# Autodesk Inventor assembly: Pok Mk3
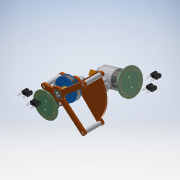
[picture p0: Inventor's stored thumbnail of the model, 180x180]
Saved by Autodesk Inventor 2018.2 (Build 222227000, 227)
## iProperties
Created: 2018-02-12
Part Number: Pok Mk3
Document SubType Name: Assembly
Designer: Moochster
Author: Moochster
## Documents named in this file (19)
- C:\Users\Moochster\OneDrive\Documents\2018 UBC\ELEC 391\Controller\CAD\Pok Mk3.iam
- C:\Users\Moochster\OneDrive\Documents\2018 UBC\ELEC 391\Controller\CAD\Brass Bushing.ipt
- C:\Users\Moochster\OneDrive\Documents\2018 UBC\ELEC 391\Controller\CAD\Rod 3-8in.ipt
- C:\Users\Moochster\OneDrive\Documents\2018 UBC\ELEC 391\Controller\CAD\R1038_ZZ_W Bearing.ipt
- C:\Users\Moochster\OneDrive\Documents\2018 UBC\ELEC 391\Controller\CAD\Yaw Platform Top.ipt
- C:\Users\Moochster\OneDrive\Documents\2018 UBC\ELEC 391\Controller\CAD\Pok Mk3\Design Accelerator\Synchronous Belts Transmission2.iam
- C:\Users\Moochster\OneDrive\Documents\2018 UBC\ELEC 391\Controller\CAD\Pok Header Mount.ipt
- C:\Users\Moochster\OneDrive\Documents\2018 UBC\ELEC 391\Controller\CAD\JD5B-2655W-R.ipt
- C:\Users\Moochster\OneDrive\Documents\2018 UBC\ELEC 391\Controller\CAD\Pok Default Pitch Motor Mount.ipt
- C:\Users\Moochster\OneDrive\Documents\2018 UBC\ELEC 391\Controller\CAD\Laser Mount.ipt
- C:\Users\Moochster\Documents\Inventor\Content Center Files\R2018\en-US\AS 1110\AS 1110 - M3 x 20.ipt
- C:\Users\Moochster\Documents\Inventor\Content Center Files\R2018\en-US\AS 1112 (2)\AS 1112 - M3  Type 5.ipt
- C:\Users\Moochster\Documents\Inventor\Content Center Files\R2018\en-US\CNS 5050\CNS 5050 - A - 3.2 8.ipt
- C:\Users\Moochster\Documents\Inventor\Content Center Files\R2018\en-US\ANSI B18.3.1M(1)\ANSI B18.3.1M - M1.6x0.35 x 3(2).ipt
- C:\Users\Moochster\OneDrive\Documents\2018 UBC\ELEC 391\Controller\CAD\Pok Mk3 Base.ipt
- C:\Users\Moochster\OneDrive\Documents\2018 UBC\ELEC 391\Controller\CAD\Pok Mk3 Support.ipt
- C:\Users\Moochster\OneDrive\Documents\2018 UBC\ELEC 391\Controller\CAD\Encoder Wheel (G16).ipt
- C:\Users\Moochster\OneDrive\Documents\2018 UBC\ELEC 391\Controller\CAD\Shaft Encoder Adapter.ipt
- C:\Users\Moochster\OneDrive\Documents\2018 UBC\ELEC 391\Controller\CAD\GP1A52HRJ00F (Large slot detector).ipt
## Components (34 placed, 18 different names)
1. Brass Bushing:1 — Mate:4, Flush:3, Mate:9
2. Brass Bushing:2 — Mate:3, Mate:8, Mate:31
3. Rod 3-8in:1 — Mate:1, Mate:2, Mate:3, Mate:4, Flush:1, Mate:6, Mate:10, Mate:23, Mate:24, Flush:6
4. R1038_ZZ_W Bearing:1 — Mate:1, Flush:1, Mate:8
5. R1038_ZZ_W Bearing:2 — Mate:2, Mate:5, Flush:2
6. Yaw Platform Top:1 — Mate:5, Flush:2, Flush:3, Mate:11, Angle:1
7. Synchronous Belts Transmission:1 [sub-assembly] — Mate:6, Mate:9, Mate:31, Mate:33
8. Pok Header Mount:1 — Mate:10, Mate:11, Mate:12, Flush:4, Mate:19, Mate:20, Mate:21
9. R1038_ZZ_W Bearing:3 — Mate:12, Flush:4
10. JD5B-2655W-R:1 — Mate:17, Mate:18, Mate:22, Flush:5, Angle:2, Tangent:1, Tangent:2, Mate:34, Mate:38
11. Laser Mount:1 — Mate:17, Mate:18
12. Pok Default Pitch Motor Mount:1 — Mate:19, Mate:20, Mate:21, Mate:22, Flush:5, Mate:25, Insert:1, Insert:3, Insert:5, Insert:7, Angle:2, Mate:26, Mate:27
13. AS 1110 - Metric M3 x 20:1 — Mate:25, Insert:2
14. AS 1110 - Metric M3 x 20:2 — Insert:6
15. CNS 5050 A - 3.2:4 — Insert:7, Insert:8
16. CNS 5050 A - 3.2:2 — Insert:5, Insert:6
17. CNS 5050 A - 3.2:3 — Insert:3, Insert:4
18. CNS 5050 A - 3.2:1 — Insert:1, Insert:2
19. AS 1112 (2) - Metric M3  Type 5:1 — Insert:8
20. AS 1112 (2) - Metric M3  Type 5:2 — Insert:4
21. Broached Socket Head Cap Screw - Metric M1.6x0.35 x 3:1 — Mate:26, Tangent:1
22. Broached Socket Head Cap Screw - Metric M1.6x0.35 x 3:2 — Mate:27, Tangent:2
23. Pok Mk3 Base:1 — Flush:6, Mate:28, Flush:7, Mate:29, Flush:8, Mate:30, Flush:9
24. Pok Mk3 Support:1 — Mate:28, Flush:7
25. Pok Mk3 Support:2 — Mate:30, Flush:9
26. Pok Mk3 Support:3 — Mate:29, Flush:8
27. JD5B-2655W-R:2 — Mate:32, Mate:33
28. Encoder Wheel (G16):1 — Mate:32
29. Encoder Wheel (G16):2 — Mate:35, Mate:36, Mate:37
30. Shaft Encoder Adapter:1 — Mate:34, Mate:35, Mate:36, Mate:37, Mate:38
31. GP1A52HRJ00F (Large slot detector):1
32. GP1A52HRJ00F (Large slot detector):2
33. GP1A52HRJ00F (Large slot detector):3
34. GP1A52HRJ00F (Large slot detector):4
## Relationships (54: Mate 33, Flush 9, Insert 8, Angle 2, Tangent 2)
- Mate:1: Rod 3-8in:1 ↔ R1038_ZZ_W Bearing:1
- Mate:2: Rod 3-8in:1 ↔ R1038_ZZ_W Bearing:2
- Mate:3: Brass Bushing:2 ↔ Rod 3-8in:1
- Mate:4: Brass Bushing:1 ↔ Rod 3-8in:1
- Flush:1: Rod 3-8in:1 ↔ R1038_ZZ_W Bearing:1
- Mate:5: R1038_ZZ_W Bearing:2 ↔ Yaw Platform Top:1
- Flush:2: R1038_ZZ_W Bearing:2 ↔ Yaw Platform Top:1
- Mate:6: Rod 3-8in:1 ↔ Synchronous Belts Transmission:1
- Mate:8 (0.1 mm): Brass Bushing:2 ↔ R1038_ZZ_W Bearing:1
- Flush:3 (0.1 mm): Brass Bushing:1 ↔ Yaw Platform Top:1
- Mate:9 (0.1 mm): Brass Bushing:1 ↔ Synchronous Belts Transmission:1
- Mate:10: Rod 3-8in:1 ↔ Pok Header Mount:1
- Mate:11 (0.2 mm): Yaw Platform Top:1 ↔ Pok Header Mount:1
- Mate:12: Pok Header Mount:1 ↔ R1038_ZZ_W Bearing:3
- Flush:4 (1 mm): Pok Header Mount:1 ↔ R1038_ZZ_W Bearing:3
- Mate:17: JD5B-2655W-R:1 ↔ Laser Mount:1
- Mate:18 (1 mm): JD5B-2655W-R:1 ↔ Laser Mount:1
- Mate:19: Pok Header Mount:1 ↔ Pok Default Pitch Motor Mount:1
- Mate:20: Pok Header Mount:1 ↔ Pok Default Pitch Motor Mount:1
- Mate:21 (0.1 mm): Pok Header Mount:1 ↔ Pok Default Pitch Motor Mount:1
- Mate:22: JD5B-2655W-R:1 ↔ Pok Default Pitch Motor Mount:1
- Mate:23: Rod 3-8in:1
- Mate:24: Rod 3-8in:1
- Angle:1 (0 deg): Yaw Platform Top:1
- Flush:5 (-10 mm): JD5B-2655W-R:1 ↔ Pok Default Pitch Motor Mount:1
- Mate:25: Pok Default Pitch Motor Mount:1 ↔ AS 1110 - Metric M3 x 20:1
- Insert:1: Pok Default Pitch Motor Mount:1 ↔ CNS 5050 A - 3.2:1
- Insert:2: AS 1110 - Metric M3 x 20:1 ↔ CNS 5050 A - 3.2:1
- Insert:3: Pok Default Pitch Motor Mount:1 ↔ CNS 5050 A - 3.2:3
- Insert:4: CNS 5050 A - 3.2:3 ↔ AS 1112 (2) - Metric M3  Type 5:2
- Insert:5: Pok Default Pitch Motor Mount:1 ↔ CNS 5050 A - 3.2:2
- Insert:6: AS 1110 - Metric M3 x 20:2 ↔ CNS 5050 A - 3.2:2
- Insert:7: Pok Default Pitch Motor Mount:1 ↔ CNS 5050 A - 3.2:4
- Insert:8: CNS 5050 A - 3.2:4 ↔ AS 1112 (2) - Metric M3  Type 5:1
- Angle:2 (180 deg): JD5B-2655W-R:1 ↔ Pok Default Pitch Motor Mount:1
- Mate:26: Pok Default Pitch Motor Mount:1 ↔ Broached Socket Head Cap Screw - Metric M1.6x0.35 x 3:1
- Tangent:1: JD5B-2655W-R:1 ↔ Broached Socket Head Cap Screw - Metric M1.6x0.35 x 3:1
- Mate:27: Pok Default Pitch Motor Mount:1 ↔ Broached Socket Head Cap Screw - Metric M1.6x0.35 x 3:2
- Tangent:2: JD5B-2655W-R:1 ↔ Broached Socket Head Cap Screw - Metric M1.6x0.35 x 3:2
- Flush:6: Rod 3-8in:1 ↔ Pok Mk3 Base:1
- Mate:28: Pok Mk3 Base:1 ↔ Pok Mk3 Support:1
- Flush:7: Pok Mk3 Base:1 ↔ Pok Mk3 Support:1
- Mate:29: Pok Mk3 Base:1 ↔ Pok Mk3 Support:3
- Flush:8: Pok Mk3 Base:1 ↔ Pok Mk3 Support:3
- Mate:30: Pok Mk3 Base:1 ↔ Pok Mk3 Support:2
- Flush:9: Pok Mk3 Base:1 ↔ Pok Mk3 Support:2
- Mate:31 (0.1 mm): Brass Bushing:2 ↔ Synchronous Belts Transmission:1
- Mate:32: JD5B-2655W-R:2 ↔ Encoder Wheel (G16):1
- Mate:33: Synchronous Belts Transmission:1 ↔ JD5B-2655W-R:2
- Mate:34: JD5B-2655W-R:1 ↔ Shaft Encoder Adapter:1
- Mate:35: Encoder Wheel (G16):2 ↔ Shaft Encoder Adapter:1
- Mate:36: Encoder Wheel (G16):2 ↔ Shaft Encoder Adapter:1
- Mate:37: Encoder Wheel (G16):2 ↔ Shaft Encoder Adapter:1
- Mate:38 (0.25 mm): JD5B-2655W-R:1 ↔ Shaft Encoder Adapter:1
